# Autodesk Inventor assembly: Serov_with_arm
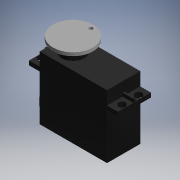
[picture p0: Inventor's stored thumbnail of the model, 180x180]
Saved by Autodesk Inventor 2017 (Build 210142000, 142)
## iProperties
Part Number: Serov_with_arm
Document SubType Name: Assembly
Designer: alex-
Author: alex-
## Documents named in this file (3)
- D:\Alexander Miller\Documents\Git\Hexapod\3DParts\Serov_with_arm.iam
- D:\Alexander Miller\Documents\Git\Hexapod\3DParts\Servo.ipt
- D:\Alexander Miller\Documents\Git\Hexapod\3DParts\Servo_arm.ipt
## Components (2 placed, 2 different names)
1. Servo:1 — Rotational:1, Flush:1, Flush:2, Flush:3
2. Servo_arm:1 — Rotational:1
## Relationships (4: Flush 3, RevoluteJoint 1)
- Rotational:1 [RevoluteJoint]: Servo:1 ↔ Servo_arm:1
- Flush:1: Servo:1
- Flush:2: Servo:1
- Flush:3: Servo:1
